# Autodesk Inventor assembly: vraie_finale
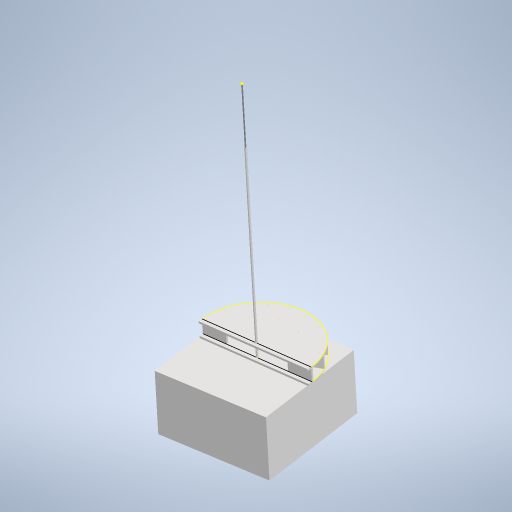
[picture p0: Inventor's stored thumbnail of the model, 512x512]
Saved by Autodesk Inventor 2023 (Build 270158000, 158)
## iProperties
Created: 2023-04-24
Part Number: vraie_finale
Document SubType Name: Assembly
Designer: Julia
Author: Julia
## Documents named in this file (7)
- C:\Users\Julia\OneDrive\Bureau\PIE\vraie_finale.iam
- C:\Users\Julia\OneDrive\Bureau\PIE\bloc percé.ipt
- C:\Users\Julia\OneDrive\Bureau\PIE\plaque dessus.ipt
- C:\Users\Julia\OneDrive\Bureau\PIE\tige filetée.ipt
- C:\Users\Julia\OneDrive\Bureau\PIE\tube acier.ipt
- C:\Users\Julia\OneDrive\Bureau\PIE\plaque de separation.ipt
- C:\Users\Julia\OneDrive\Bureau\PIE\barre plaque.ipt
## Components (35 placed, 6 different names)
1. bloc percé:1 — Placage:1, Placage:2
2. plaque dessus:1 — Placage:1, Placage:2, Placage:3, Rotation:1, Placage:5, Placage:7, Placage:8, Placage:9, Placage:10, Placage:11, Logement:1, Logement:2, Logement:3, Logement:4, Logement:5, Logement:6, Logement:7, Logement:8, Logement:9, Logement:10, Logement:11, Logement:12, Logement:13, Logement:14, Logement:15, Logement:16, Logement:17, Placage:14, Placage:17, Placage:18, Placage:20, Placage:22, Placage:25, Placage:29, Placage:30, Placage:32, Placage:34
3. tige filetée:1 — Placage:3, Placage:4
4. tube acier:1 — Placage:4, Rotation:1
5. plaque de separation:2 — Placage:15, Placage:17
6. plaque de separation:3 — Placage:26, Placage:30
7. plaque de separation:4 — Placage:21, Placage:22
8. plaque de separation:5 — Placage:23, Placage:24, Placage:25, Placage:36
9. plaque de separation:6 — Placage:19, Placage:20
10. plaque de separation:7 — Placage:16, Placage:18
11. plaque de separation:10 — Placage:12, Placage:13, Placage:14, Placage:35
12. barre plaque:1 — Placage:7, Placage:11, Placage:12
13. barre plaque:2 — Placage:5, Placage:10, Placage:13
14. barre plaque:3 — Placage:8, Placage:9
15. barre plaque:4 — Logement:4, Placage:19
16. barre plaque:5 — Logement:5
17. barre plaque:6 — Logement:6, Placage:21
18. barre plaque:7 — Logement:2, Placage:16
19. barre plaque:8 — Logement:1, Placage:15
20. barre plaque:9 — Logement:3
21. barre plaque:10 — Logement:7
22. barre plaque:11 — Logement:11
23. barre plaque:12 — Logement:15
24. barre plaque:13 — Logement:14
25. barre plaque:14 — Logement:12, Placage:26
26. barre plaque:15 — Logement:13, Placage:28
27. barre plaque:16 — Logement:16, Placage:23
28. barre plaque:17 — Logement:17, Placage:24
29. barre plaque:18 — Logement:10, Placage:31
30. barre plaque:19 — Logement:9
31. barre plaque:20 — Logement:8, Placage:33
32. plaque de separation:11 — Placage:28, Placage:29
33. plaque de separation:12 — Placage:31, Placage:32
34. plaque de separation:13 — Placage:33, Placage:34
35. plaque dessus:2 — Placage:35, Placage:36
## Relationships (52: Mate 34, Insert 17, RevoluteJoint 1)
- Placage:1 [Mate]: bloc percé:1 ↔ plaque dessus:1
- Placage:2 [Mate]: bloc percé:1 ↔ plaque dessus:1
- Placage:3 [Mate]: plaque dessus:1 ↔ tige filetée:1
- Placage:4 [Mate]: tige filetée:1 ↔ tube acier:1
- Rotation:1 [RevoluteJoint]: plaque dessus:1 ↔ tube acier:1
- Placage:5 [Mate]: plaque dessus:1 ↔ barre plaque:2
- Placage:7 [Mate]: plaque dessus:1 ↔ barre plaque:1
- Placage:8 [Mate]: plaque dessus:1 ↔ barre plaque:3
- Placage:9 [Mate]: plaque dessus:1 ↔ barre plaque:3
- Placage:10 [Mate]: plaque dessus:1 ↔ barre plaque:2
- Placage:11 [Mate]: plaque dessus:1 ↔ barre plaque:1
- Logement:1 [Insert]: plaque dessus:1 ↔ barre plaque:8
- Logement:2 [Insert]: plaque dessus:1 ↔ barre plaque:7
- Logement:3 [Insert]: plaque dessus:1 ↔ barre plaque:9
- Logement:4 [Insert]: plaque dessus:1 ↔ barre plaque:4
- Logement:5 [Insert]: plaque dessus:1 ↔ barre plaque:5
- Logement:6 [Insert]: plaque dessus:1 ↔ barre plaque:6
- Logement:7 [Insert]: plaque dessus:1 ↔ barre plaque:10
- Logement:8 [Insert]: plaque dessus:1 ↔ barre plaque:20
- Logement:9 [Insert]: plaque dessus:1 ↔ barre plaque:19
- Logement:10 [Insert]: plaque dessus:1 ↔ barre plaque:18
- Logement:11 [Insert]: plaque dessus:1 ↔ barre plaque:11
- Logement:12 [Insert]: plaque dessus:1 ↔ barre plaque:14
- Logement:13 [Insert]: plaque dessus:1 ↔ barre plaque:15
- Logement:14 [Insert]: plaque dessus:1 ↔ barre plaque:13
- Logement:15 [Insert]: plaque dessus:1 ↔ barre plaque:12
- Logement:16 [Insert]: plaque dessus:1 ↔ barre plaque:16
- Logement:17 [Insert]: plaque dessus:1 ↔ barre plaque:17
- Placage:12 [Mate]: plaque de separation:10 ↔ barre plaque:1
- Placage:13 [Mate]: plaque de separation:10 ↔ barre plaque:2
- Placage:14 [Mate]: plaque dessus:1 ↔ plaque de separation:10
- Placage:15 [Mate]: plaque de separation:2 ↔ barre plaque:8
- Placage:16 [Mate]: plaque de separation:7 ↔ barre plaque:7
- Placage:17 [Mate]: plaque dessus:1 ↔ plaque de separation:2
- Placage:18 [Mate]: plaque dessus:1 ↔ plaque de separation:7
- Placage:19 [Mate]: plaque de separation:6 ↔ barre plaque:4
- Placage:20 [Mate]: plaque dessus:1 ↔ plaque de separation:6
- Placage:21 [Mate]: plaque de separation:4 ↔ barre plaque:6
- Placage:22 [Mate]: plaque dessus:1 ↔ plaque de separation:4
- Placage:23 [Mate]: plaque de separation:5 ↔ barre plaque:16
- Placage:24 [Mate]: plaque de separation:5 ↔ barre plaque:17
- Placage:25 [Mate]: plaque dessus:1 ↔ plaque de separation:5
- Placage:26 [Mate]: plaque de separation:3 ↔ barre plaque:14
- Placage:28 [Mate]: barre plaque:15 ↔ plaque de separation:11
- Placage:29 [Mate]: plaque dessus:1 ↔ plaque de separation:11
- Placage:30 [Mate]: plaque dessus:1 ↔ plaque de separation:3
- Placage:31 [Mate]: barre plaque:18 ↔ plaque de separation:12
- Placage:32 [Mate]: plaque dessus:1 ↔ plaque de separation:12
- Placage:33 [Mate]: barre plaque:20 ↔ plaque de separation:13
- Placage:34 [Mate]: plaque dessus:1 ↔ plaque de separation:13
- Placage:35 [Mate]: plaque de separation:10 ↔ plaque dessus:2
- Placage:36 [Mate]: plaque de separation:5 ↔ plaque dessus:2
